# Autodesk Inventor assembly: Robot
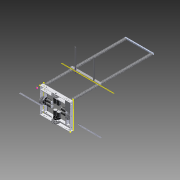
[picture p0: Inventor's stored thumbnail of the model, 180x180]
Saved by Autodesk Inventor 2015 (Build 190159000, 159)
## iProperties
Created: 2015-01-10
Part Number: Robot
Document SubType Name: Assembly
Designer: jhirshland1
Mass: 11000.2 g
Surface Area: 53233.2 cm^2
Volume: 11000.2 cm^3
Density: 1 g/cm^3
Author: jhirshland1
## Documents named in this file (9)
- C:\Users\jhirshland1\Inventor\HWRobot2015CAD\Chassis\Chassis.iam
- C:\Users\jhirshland1\Inventor\HWRobot2015CAD\FRCKOP2015\Drive Base\am-2951 AM14U2 Outside Sheet.ipt
- C:\Users\jhirshland1\Inventor\HWRobot2015CAD\FRCKOP2015\Drive Base\am-2951 AM14U2 Ouside 23i.ipt
- C:\Users\jhirshland1\Inventor\HWRobot2015CAD\FRCKOP2015\Drive Base\am-2952 AM14U2 Inside Sheet.ipt
- C:\Users\jhirshland1\Inventor\HWRobot2015CAD\FRCKOP2015\AndyMark\WheelAssembly.iam
- C:\Users\jhirshland1\Inventor\HWRobot2015CAD\FRCKOP2015\AndyMark\SecondWheelAssembl.iam
- C:\Users\jhirshland1\Inventor\HWRobot2015CAD\Whole Elevator Static Structure.iam
- C:\Users\jhirshland1\Inventor\HWRobot2015CAD\Aluminum Final.ipt
- C:\Users\jhirshland1\Inventor\HWRobot2015CAD\FRCKOP2015\McMaster\47065T125.ipt
## Components (17 placed, 8 different names)
1. am-2951 AM14U2 Outside Sheet:1 — Mate:5, Mate:8, Flush:16, Flush:19, Flush:21, Flush:22, Flush:27
2. am-2951 AM14U2 Outside Sheet:2 — Mate:22, Flush:13, Flush:14, Flush:25
3. am-2951 AM14U2 Ouside 23i:1 — Mate:5, Mate:19, Flush:16, Flush:17, Flush:18, Flush:19, Flush:23, Insert:5, Insert:6, Insert:9, Insert:10
4. am-2951 AM14U2 Ouside 23i:2 — Mate:8, Mate:13, Mate:17, Mate:21, Mate:22, Flush:13, Flush:14, Flush:21, Flush:24, Insert:11, Insert:12
5. am-2952 AM14U2 Inside Sheet:1 — Mate:17, Mate:18, Mate:20, Flush:11, Flush:12, Flush:25
6. am-2952 AM14U2 Inside Sheet:2 — Mate:13, Insert:3, Insert:4, Flush:17, Flush:18, Flush:20, Flush:22, Flush:23, Flush:26, Flush:27
7. WheelAssembly:1 [sub-assembly]
8. WheelAssembly:2 [sub-assembly] — Insert:3, Insert:4
9. SecondWheelAssembl:1 [sub-assembly] — Mate:18, Mate:19, Flush:12, Flush:20
10. SecondWheelAssembl:2 [sub-assembly] — Mate:20, Flush:11, Mate:21, Flush:24, Flush:26
11. Whole Elevator Static Structure:1 [sub-assembly] — Insert:7, Insert:8, Flush:28, Mate:23, Tangent:1, Flush:29, Tangent:2, Mate:24, Mate:25
12. Aluminum Final:1 — Insert:7, Insert:8
13. Aluminum Final:2 — Insert:5, Insert:6
14. 47065T125:1 — Flush:28, Mate:23, Tangent:1
15. 47065T125:2 — Flush:29, Tangent:2, Mate:24
16. Aluminum Final:3 — Insert:9, Insert:10, Mate:25
17. Aluminum Final:4 — Insert:11, Insert:12
## Relationships (44: Flush 18, Mate 12, Insert 12, Tangent 2)
- Mate:5: am-2951 AM14U2 Outside Sheet:1 ↔ am-2951 AM14U2 Ouside 23i:1
- Mate:8: am-2951 AM14U2 Outside Sheet:1 ↔ am-2951 AM14U2 Ouside 23i:2
- Mate:13: am-2951 AM14U2 Ouside 23i:2 ↔ am-2952 AM14U2 Inside Sheet:2
- Mate:17: am-2951 AM14U2 Ouside 23i:2 ↔ am-2952 AM14U2 Inside Sheet:1
- [Insert]: am-2952 AM14U2 Inside Sheet:1 ↔ WheelAssembly:1
- [Insert]: am-2952 AM14U2 Inside Sheet:1 ↔ WheelAssembly:1
- Insert:3: am-2952 AM14U2 Inside Sheet:2 ↔ WheelAssembly:2
- Insert:4: am-2952 AM14U2 Inside Sheet:2 ↔ WheelAssembly:2
- Mate:18: am-2952 AM14U2 Inside Sheet:1 ↔ SecondWheelAssembl:1
- Mate:19 (85.09 mm): am-2951 AM14U2 Ouside 23i:1 ↔ SecondWheelAssembl:1
- Mate:20: am-2952 AM14U2 Inside Sheet:1 ↔ SecondWheelAssembl:2
- Flush:11: am-2952 AM14U2 Inside Sheet:1 ↔ SecondWheelAssembl:2
- Mate:21 (85.09 mm): am-2951 AM14U2 Ouside 23i:2 ↔ SecondWheelAssembl:2
- Flush:12: am-2952 AM14U2 Inside Sheet:1 ↔ SecondWheelAssembl:1
- Mate:22: am-2951 AM14U2 Outside Sheet:2 ↔ am-2951 AM14U2 Ouside 23i:2
- Flush:13: am-2951 AM14U2 Outside Sheet:2 ↔ am-2951 AM14U2 Ouside 23i:2
- Flush:14: am-2951 AM14U2 Outside Sheet:2 ↔ am-2951 AM14U2 Ouside 23i:2
- Flush:16: am-2951 AM14U2 Outside Sheet:1 ↔ am-2951 AM14U2 Ouside 23i:1
- Flush:17: am-2951 AM14U2 Ouside 23i:1 ↔ am-2952 AM14U2 Inside Sheet:2
- Flush:18: am-2951 AM14U2 Ouside 23i:1 ↔ am-2952 AM14U2 Inside Sheet:2
- Flush:19: am-2951 AM14U2 Outside Sheet:1 ↔ am-2951 AM14U2 Ouside 23i:1
- Flush:20: am-2952 AM14U2 Inside Sheet:2 ↔ SecondWheelAssembl:1
- Flush:21: am-2951 AM14U2 Outside Sheet:1 ↔ am-2951 AM14U2 Ouside 23i:2
- Flush:22: am-2951 AM14U2 Outside Sheet:1 ↔ am-2952 AM14U2 Inside Sheet:2
- Flush:23: am-2951 AM14U2 Ouside 23i:1 ↔ am-2952 AM14U2 Inside Sheet:2
- Flush:24: am-2951 AM14U2 Ouside 23i:2 ↔ SecondWheelAssembl:2
- Flush:25: am-2951 AM14U2 Outside Sheet:2 ↔ am-2952 AM14U2 Inside Sheet:1
- Flush:26: am-2952 AM14U2 Inside Sheet:2 ↔ SecondWheelAssembl:2
- Flush:27: am-2951 AM14U2 Outside Sheet:1 ↔ am-2952 AM14U2 Inside Sheet:2
- Insert:5: am-2951 AM14U2 Ouside 23i:1 ↔ Aluminum Final:2
- Insert:6: am-2951 AM14U2 Ouside 23i:1 ↔ Aluminum Final:2
- Insert:7 (25.4 mm): Whole Elevator Static Structure:1 ↔ Aluminum Final:1
- Insert:8 (25.4 mm): Whole Elevator Static Structure:1 ↔ Aluminum Final:1
- Flush:28: Whole Elevator Static Structure:1 ↔ 47065T125:1
- Mate:23: Whole Elevator Static Structure:1 ↔ 47065T125:1
- Tangent:1: Whole Elevator Static Structure:1 ↔ 47065T125:1
- Flush:29: Whole Elevator Static Structure:1 ↔ 47065T125:2
- Tangent:2: Whole Elevator Static Structure:1 ↔ 47065T125:2
- Mate:24: Whole Elevator Static Structure:1 ↔ 47065T125:2
- Insert:9: am-2951 AM14U2 Ouside 23i:1 ↔ Aluminum Final:3
- Insert:10: am-2951 AM14U2 Ouside 23i:1 ↔ Aluminum Final:3
- Insert:11: am-2951 AM14U2 Ouside 23i:2 ↔ Aluminum Final:4
- Insert:12: am-2951 AM14U2 Ouside 23i:2 ↔ Aluminum Final:4
- Mate:25: Whole Elevator Static Structure:1 ↔ Aluminum Final:3
